# Autodesk Inventor assembly: linear_guide
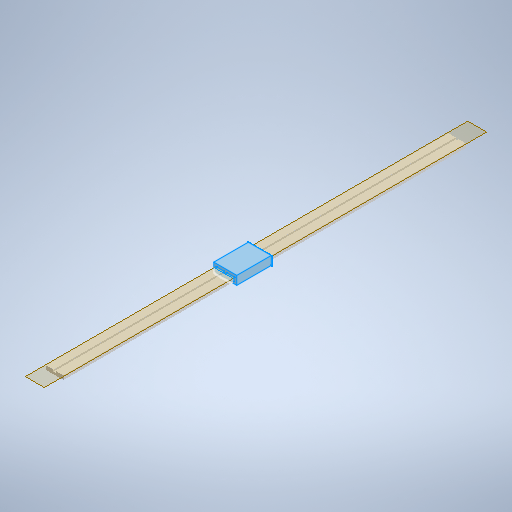
[picture p0: Inventor's stored thumbnail of the model, 512x512]
Saved by Autodesk Inventor 2025.1 (Build 291241000, 241)
## iProperties
Created: 2024-11-25
Part Number: linear_guide
Document SubType Name: Assembly
Designer: dell
Author: dell
## Documents named in this file (3)
- D:\creap\prot_tonbo\linear_guide.iam
- D:\creap\prot_tonbo\linia.ipt
- D:\creap\prot_tonbo\guide.ipt
## Components (2 placed, 2 different names)
1. linia:1 — スライダ:1
2. guide:1 — スライダ:1
## Relationships (1: TranslationJoint 1)
- スライダ:1 [TranslationJoint]: linia:1 ↔ guide:1
